# Autodesk Inventor assembly: gantry_frame
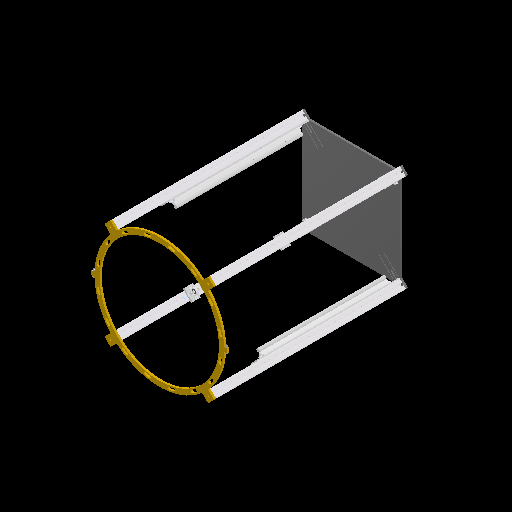
[picture p0: Inventor's stored thumbnail of the model, 512x512]
Saved by Autodesk Inventor 2026.1 (Build 301233000, 233)
## iProperties
Created: 2025-09-18
Part Number: gantry_frame
Document SubType Name: Assembly
Designer: drago
Author: drago
## Documents named in this file (6)
- C:\Users\drago\Desktop\_QIST4500_Multidisciplinary_Team_Project\Proteox MX magnet positioner CAD\gantry_frame\gantry_frame.iam
- C:\Users\drago\Desktop\_QIST4500_Multidisciplinary_Team_Project\Proteox MX magnet positioner CAD\gantry_frame\square_bar.ipt
- C:\Users\drago\Desktop\_QIST4500_Multidisciplinary_Team_Project\Proteox MX magnet positioner CAD\gantry_frame\base_plate.ipt
- C:\Users\drago\Desktop\_QIST4500_Multidisciplinary_Team_Project\Proteox MX magnet positioner CAD\z_rail\z_rail.iam
- C:\Users\drago\Desktop\_QIST4500_Multidisciplinary_Team_Project\Proteox MX magnet positioner CAD\z_translator\z_translator.iam
- C:\Users\drago\Desktop\_QIST4500_Multidisciplinary_Team_Project\Proteox MX magnet positioner CAD\gantry_frame\full_ring.iam
## Components (10 placed, 5 different names)
1. full_ring:1 [sub-assembly] — Mate:60, Mate:61, Mate:62
2. base_plate:1 — Mate:45, Angle:2, Mate:46, Mate:47, Mate:48, Mate:49, Mate:52, Mate:53, Mate:54, Mate:55, Mate:58, Mate:59
3. z_rail:1 [sub-assembly] — Mate:48, Mate:50, Mate:53
4. z_rail:2 [sub-assembly] — Mate:49, Mate:51, Mate:52
5. z_translator:1 [sub-assembly] — Mate:54, Mate:56, Mate:59
6. z_translator:2 [sub-assembly] — Mate:55, Mate:57, Mate:58
7. square_bar:1 — Angle:1, Mate:46, Mate:47, Mate:51
8. square_bar:2 — Mate:56
9. square_bar:3 — Mate:50, Mate:62
10. square_bar:4 — Mate:57
## Component patterns: (4 elements, first: square_bar:1)
## Relationships (20: Mate 18, Angle 2)
- Angle:1 (45 deg): square_bar:1
- Mate:45: base_plate:1
- Angle:2 (45 deg): base_plate:1
- Mate:46: base_plate:1 ↔ square_bar:1
- Mate:47: base_plate:1 ↔ square_bar:1
- Mate:48: base_plate:1 ↔ z_rail:1
- Mate:49: base_plate:1 ↔ z_rail:2
- Mate:50: z_rail:1 ↔ square_bar:3
- Mate:51: z_rail:2 ↔ square_bar:1
- Mate:52: base_plate:1 ↔ z_rail:2
- Mate:53: base_plate:1 ↔ z_rail:1
- Mate:54: base_plate:1 ↔ z_translator:1
- Mate:55: base_plate:1 ↔ z_translator:2
- Mate:56: z_translator:1 ↔ square_bar:2
- Mate:57: z_translator:2 ↔ square_bar:4
- Mate:58: base_plate:1 ↔ z_translator:2
- Mate:59: base_plate:1 ↔ z_translator:1
- Mate:60: full_ring:1
- Mate:61: full_ring:1
- Mate:62: full_ring:1 ↔ square_bar:3
